# Autodesk Inventor assembly: SBR12UU
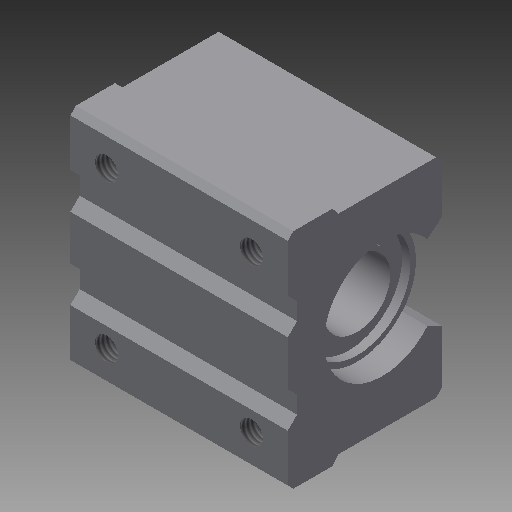
[picture p0: Inventor's stored thumbnail of the model, 512x512]
Saved by Autodesk Inventor 2018 (Build 220112000, 112)
## iProperties
Created: 2018-07-23
Part Number: SBR12UU
Material: Genérico
Document SubType Name: Assembly
Designer: Usuario
Mass: 31.9458 g
Surface Area: 161.318 cm^2
Volume: 31.9458 cm^3
Density: 1 g/cm^3
Author: Usuario
## Documents named in this file (4)
- C:\Users\Usuario\Desktop\Estação BGA\Peças 3D\SBR12UU.iam
- C:\Users\Usuario\Desktop\Estação BGA\Peças 3D\rolamento_linear_lm12uu.iam.ipt
- C:\Users\Usuario\Desktop\Estação BGA\Peças 3D\PilowBlockAberto.ipt
- rolamento_linear_lm12uu.iam
## Components (2 placed, 2 different names)
1. rolamento_linear_lm12uu.iam:1 — Alinhamento:1, Coincidência:1
2. PilowBlockAberto:1 — Alinhamento:1, Coincidência:1
## Relationships (2: Flush 1, Mate 1)
- Alinhamento:1 [Flush] (4.5 mm): rolamento_linear_lm12uu.iam:1 ↔ PilowBlockAberto:1
- Coincidência:1 [Mate]: rolamento_linear_lm12uu.iam:1 ↔ PilowBlockAberto:1
